# Autodesk Inventor assembly: DriveTrain_FrameAssembly
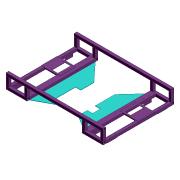
[picture p0: Inventor's stored thumbnail of the model, 180x180]
Saved by Autodesk Inventor 2012 (Build 160160000, 160)
## iProperties
Created: 2012-01-07
Part Number: DriveTrain_FrameAssembly
Document SubType Name: Assembly
Designer: JesseK
Mass: 6410.77 g
Surface Area: 17866.8 cm^2
Volume: 2365.6 cm^3
Density: 2.71 g/cm^3
Author: JesseK
## Documents named in this file (10)
- Z:\UserData\Documents\Inventor\team1885frc\Robot2012\DriveTrain\DriveTrain_FrameAssembly.iam
- Z:\UserData\Documents\Inventor\team1885frc\Robot2012\DriveTrain\DriveTrain_SideRail.ipt
- Z:\UserData\Documents\Inventor\team1885frc\Robot2012\DriveTrain\FrontBumperRail.ipt
- Z:\UserData\Documents\Inventor\team1885frc\Robot2012\DriveTrain\Frame_SideRail_Inner_2x1.ipt
- Z:\UserData\Documents\Inventor\team1885frc\Robot2012\DriveTrain\WheelBlockMount.ipt
- Z:\UserData\Documents\Inventor\team1885frc\Robot2012\DriveTrain\DriveTrain_MotorMount.ipt
- Z:\UserData\Documents\Inventor\team1885frc\Robot2012\DriveTrain\Frame_LongCrossMember.ipt
- Z:\UserData\Documents\Inventor\team1885frc\Robot2012\DriveTrain\Frame_FrontVerticalSupport_forFrontCrossbar.ipt
- Z:\UserData\Documents\Inventor\team1885frc\Robot2012\DriveTrain\Frame_BottomLeftMountPlate.ipt
- Z:\UserData\Documents\Inventor\team1885frc\Robot2012\DriveTrain\Frame_BottomRightMountPlate.ipt
## Components (30 placed, 9 different names)
1. DriveTrain_SideRail:1 — Flush:1, Flush:2, Mate:1, Flush:4, Mate:2, Mate:11, Mate:18, Mate:19, Mate:20, Mate:23, Mate:24, Mate:140
2. Frame_SideRail_Inner_2x1:1 — Flush:1, Flush:2, Mate:1, Flush:3, Mate:12, Mate:17, Mate:21, Mate:22, Mate:25, Mate:26, Mate:37, Flush:21, Mate:67, Mate:68, Mate:241, Mate:242
3. FrontBumperRail:1 — Flush:3, Flush:4, Mate:2, Mate:190, Mate:191, Mate:192, Mate:193, Mate:194, Mate:199, Mate:243
4. Frame_SideRail_Inner_2x1:2 — Flush:9, Flush:10, Mate:7, Mate:10, Mate:13, Mate:15, Mate:27, Mate:28, Mate:31, Mate:32, Mate:35, Flush:20, Mate:65, Mate:228, Mate:238, Mate:239
5. FrontBumperRail:2 — Flush:9, Flush:10, Mate:7, Mate:10, Mate:141, Mate:142, Mate:172, Mate:173, Mate:174, Mate:175, Mate:176, Mate:200, Mate:240
6. DriveTrain_SideRail:2 — Mate:14, Mate:16, Mate:29, Mate:30, Mate:33, Mate:34, Mate:66, Mate:141, Mate:142, Mate:143
7. WheelBlockMount:1 — Mate:16, Mate:33, Mate:34
8. WheelBlockMount:2 — Mate:17, Mate:21, Mate:22
9. WheelBlockMount:3 — Mate:18, Mate:19, Mate:20
10. WheelBlockMount:4 — Mate:13, Mate:27, Mate:28
11. WheelBlockMount:5 — Mate:11, Mate:23, Mate:24
12. WheelBlockMount:6 — Mate:12, Mate:25, Mate:26
13. WheelBlockMount:7 — Mate:15, Mate:31, Mate:32
14. WheelBlockMount:8 — Mate:14, Mate:29, Mate:30
15. FrontBumperRail:3 — Flush:20, Mate:65, Mate:66, Mate:185, Mate:186, Mate:187, Mate:207, Mate:208, Mate:209, Mate:228
16. FrontBumperRail:4 — Flush:21, Mate:67, Mate:68, Mate:204, Mate:205, Mate:206, Mate:210, Mate:211, Mate:212
17. DriveTrain_MotorMount:1 — Mate:35, Mate:143, Mate:144
18. DriveTrain_MotorMount:2 — Mate:37, Mate:140, Mate:144
19. Frame_LongCrossMember:1 — Mate:188, Mate:189, Mate:214, Mate:237
20. Frame_LongCrossMember:2 — Mate:177, Mate:215
21. Frame_FrontVerticalSupport_forFrontCrossbar:11 — Mate:185, Mate:186, Mate:188, Mate:189, Mate:209
22. Frame_FrontVerticalSupport_forFrontCrossbar:12 — Mate:187, Mate:207, Mate:208
23. Frame_FrontVerticalSupport_forFrontCrossbar:15 — Mate:174, Mate:175, Mate:176, Mate:177
24. Frame_FrontVerticalSupport_forFrontCrossbar:16 — Mate:172, Mate:173, Mate:200, Mate:215
25. Frame_FrontVerticalSupport_forFrontCrossbar:17 — Mate:190, Mate:191, Mate:192
26. Frame_FrontVerticalSupport_forFrontCrossbar:18 — Mate:193, Mate:194, Mate:199
27. Frame_FrontVerticalSupport_forFrontCrossbar:21 — Mate:204, Mate:205, Mate:206, Mate:214, Mate:237
28. Frame_FrontVerticalSupport_forFrontCrossbar:22 — Mate:210, Mate:211, Mate:212
29. Frame_BottomLeftMountPlate:1 — Mate:238, Mate:239, Mate:240
30. Frame_BottomRightMountPlate:1 — Mate:241, Mate:242, Mate:243
## Relationships (84: Mate 76, Flush 8)
- Flush:1: DriveTrain_SideRail:1 ↔ Frame_SideRail_Inner_2x1:1
- Flush:2: DriveTrain_SideRail:1 ↔ Frame_SideRail_Inner_2x1:1
- Mate:1 (127 mm): DriveTrain_SideRail:1 ↔ Frame_SideRail_Inner_2x1:1
- Flush:3: Frame_SideRail_Inner_2x1:1 ↔ FrontBumperRail:1
- Flush:4: DriveTrain_SideRail:1 ↔ FrontBumperRail:1
- Mate:2: DriveTrain_SideRail:1 ↔ FrontBumperRail:1
- Flush:9: Frame_SideRail_Inner_2x1:2 ↔ FrontBumperRail:2
- Flush:10: Frame_SideRail_Inner_2x1:2 ↔ FrontBumperRail:2
- Mate:7: Frame_SideRail_Inner_2x1:2 ↔ FrontBumperRail:2
- Mate:10: Frame_SideRail_Inner_2x1:2 ↔ FrontBumperRail:2
- Mate:11: DriveTrain_SideRail:1 ↔ WheelBlockMount:5
- Mate:12: Frame_SideRail_Inner_2x1:1 ↔ WheelBlockMount:6
- Mate:13: Frame_SideRail_Inner_2x1:2 ↔ WheelBlockMount:4
- Mate:14: DriveTrain_SideRail:2 ↔ WheelBlockMount:8
- Mate:15: Frame_SideRail_Inner_2x1:2 ↔ WheelBlockMount:7
- Mate:16: DriveTrain_SideRail:2 ↔ WheelBlockMount:1
- Mate:17: Frame_SideRail_Inner_2x1:1 ↔ WheelBlockMount:2
- Mate:18: DriveTrain_SideRail:1 ↔ WheelBlockMount:3
- Mate:19: DriveTrain_SideRail:1 ↔ WheelBlockMount:3
- Mate:20: DriveTrain_SideRail:1 ↔ WheelBlockMount:3
- Mate:21: Frame_SideRail_Inner_2x1:1 ↔ WheelBlockMount:2
- Mate:22: Frame_SideRail_Inner_2x1:1 ↔ WheelBlockMount:2
- Mate:23: DriveTrain_SideRail:1 ↔ WheelBlockMount:5
- Mate:24: DriveTrain_SideRail:1 ↔ WheelBlockMount:5
- Mate:25: Frame_SideRail_Inner_2x1:1 ↔ WheelBlockMount:6
- Mate:26: Frame_SideRail_Inner_2x1:1 ↔ WheelBlockMount:6
- Mate:27: Frame_SideRail_Inner_2x1:2 ↔ WheelBlockMount:4
- Mate:28: Frame_SideRail_Inner_2x1:2 ↔ WheelBlockMount:4
- Mate:29: DriveTrain_SideRail:2 ↔ WheelBlockMount:8
- Mate:30: DriveTrain_SideRail:2 ↔ WheelBlockMount:8
- Mate:31: Frame_SideRail_Inner_2x1:2 ↔ WheelBlockMount:7
- Mate:32: Frame_SideRail_Inner_2x1:2 ↔ WheelBlockMount:7
- Mate:33: DriveTrain_SideRail:2 ↔ WheelBlockMount:1
- Mate:34: DriveTrain_SideRail:2 ↔ WheelBlockMount:1
- Mate:35: Frame_SideRail_Inner_2x1:2 ↔ DriveTrain_MotorMount:1
- Mate:37: Frame_SideRail_Inner_2x1:1 ↔ DriveTrain_MotorMount:2
- Flush:20: Frame_SideRail_Inner_2x1:2 ↔ FrontBumperRail:3
- Mate:65: Frame_SideRail_Inner_2x1:2 ↔ FrontBumperRail:3
- Mate:66: DriveTrain_SideRail:2 ↔ FrontBumperRail:3
- Flush:21: Frame_SideRail_Inner_2x1:1 ↔ FrontBumperRail:4
- Mate:67: Frame_SideRail_Inner_2x1:1 ↔ FrontBumperRail:4
- Mate:68: Frame_SideRail_Inner_2x1:1 ↔ FrontBumperRail:4
- Mate:140: DriveTrain_SideRail:1 ↔ DriveTrain_MotorMount:2
- Mate:141: FrontBumperRail:2 ↔ DriveTrain_SideRail:2
- Mate:142: FrontBumperRail:2 ↔ DriveTrain_SideRail:2
- Mate:143: DriveTrain_SideRail:2 ↔ DriveTrain_MotorMount:1
- Mate:144: DriveTrain_MotorMount:1 ↔ DriveTrain_MotorMount:2
- Mate:172: FrontBumperRail:2 ↔ Frame_FrontVerticalSupport_forFrontCrossbar:16
- Mate:173: FrontBumperRail:2 ↔ Frame_FrontVerticalSupport_forFrontCrossbar:16
- Mate:174: FrontBumperRail:2 ↔ Frame_FrontVerticalSupport_forFrontCrossbar:15
- Mate:175: FrontBumperRail:2 ↔ Frame_FrontVerticalSupport_forFrontCrossbar:15
- Mate:176: FrontBumperRail:2 ↔ Frame_FrontVerticalSupport_forFrontCrossbar:15
- Mate:177: Frame_LongCrossMember:2 ↔ Frame_FrontVerticalSupport_forFrontCrossbar:15
- Mate:185: FrontBumperRail:3 ↔ Frame_FrontVerticalSupport_forFrontCrossbar:11
- Mate:186: FrontBumperRail:3 ↔ Frame_FrontVerticalSupport_forFrontCrossbar:11
- Mate:187: FrontBumperRail:3 ↔ Frame_FrontVerticalSupport_forFrontCrossbar:12
- Mate:188: Frame_LongCrossMember:1 ↔ Frame_FrontVerticalSupport_forFrontCrossbar:11
- Mate:189: Frame_LongCrossMember:1 ↔ Frame_FrontVerticalSupport_forFrontCrossbar:11
- Mate:190: FrontBumperRail:1 ↔ Frame_FrontVerticalSupport_forFrontCrossbar:17
- Mate:191: FrontBumperRail:1 ↔ Frame_FrontVerticalSupport_forFrontCrossbar:17
- Mate:192: FrontBumperRail:1 ↔ Frame_FrontVerticalSupport_forFrontCrossbar:17
- Mate:193: FrontBumperRail:1 ↔ Frame_FrontVerticalSupport_forFrontCrossbar:18
- Mate:194: FrontBumperRail:1 ↔ Frame_FrontVerticalSupport_forFrontCrossbar:18
- Mate:199: FrontBumperRail:1 ↔ Frame_FrontVerticalSupport_forFrontCrossbar:18
- Mate:200: FrontBumperRail:2 ↔ Frame_FrontVerticalSupport_forFrontCrossbar:16
- Mate:204: FrontBumperRail:4 ↔ Frame_FrontVerticalSupport_forFrontCrossbar:21
- Mate:205: FrontBumperRail:4 ↔ Frame_FrontVerticalSupport_forFrontCrossbar:21
- Mate:206: FrontBumperRail:4 ↔ Frame_FrontVerticalSupport_forFrontCrossbar:21
- Mate:207: FrontBumperRail:3 ↔ Frame_FrontVerticalSupport_forFrontCrossbar:12
- Mate:208: FrontBumperRail:3 ↔ Frame_FrontVerticalSupport_forFrontCrossbar:12
- Mate:209: FrontBumperRail:3 ↔ Frame_FrontVerticalSupport_forFrontCrossbar:11
- Mate:210: FrontBumperRail:4 ↔ Frame_FrontVerticalSupport_forFrontCrossbar:22
- Mate:211: FrontBumperRail:4 ↔ Frame_FrontVerticalSupport_forFrontCrossbar:22
- Mate:212: FrontBumperRail:4 ↔ Frame_FrontVerticalSupport_forFrontCrossbar:22
- Mate:214: Frame_LongCrossMember:1 ↔ Frame_FrontVerticalSupport_forFrontCrossbar:21
- Mate:215: Frame_LongCrossMember:2 ↔ Frame_FrontVerticalSupport_forFrontCrossbar:16
- Mate:228: Frame_SideRail_Inner_2x1:2 ↔ FrontBumperRail:3
- Mate:237: Frame_LongCrossMember:1 ↔ Frame_FrontVerticalSupport_forFrontCrossbar:21
- Mate:238: Frame_SideRail_Inner_2x1:2 ↔ Frame_BottomLeftMountPlate:1
- Mate:239 (-25.4 mm): Frame_SideRail_Inner_2x1:2 ↔ Frame_BottomLeftMountPlate:1
- Mate:240: FrontBumperRail:2 ↔ Frame_BottomLeftMountPlate:1
- Mate:241: Frame_SideRail_Inner_2x1:1 ↔ Frame_BottomRightMountPlate:1
- Mate:242 (-25.4 mm): Frame_SideRail_Inner_2x1:1 ↔ Frame_BottomRightMountPlate:1
- Mate:243: FrontBumperRail:1 ↔ Frame_BottomRightMountPlate:1
